# Autodesk Inventor assembly: X_CarriageR_V2_0_Short
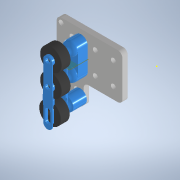
[picture p0: Inventor's stored thumbnail of the model, 180x180]
Saved by Autodesk Inventor 2021 (Build 250183000, 183)
## iProperties
Created: 2021-06-13
Part Number: X_CarriageR_V2_0_Short
Document SubType Name: Assembly
Designer: Jorian Brusind
Author: Jorian Brusind
## Documents named in this file (6)
- C:\Users\Jorian Bruslind\Documents\GitHub\PersonalProjects\HyperRail\Inventor Files\X_CarriageR_V2_0_Short.iam
- C:\Users\Jorian Bruslind\Documents\GitHub\PersonalProjects\HyperRail\Inventor Files\11mm_BearingWheel.ipt
- C:\Users\Jorian Bruslind\Documents\GitHub\PersonalProjects\HyperRail\Inventor Files\4mm_Roller_Spacer_simple.ipt
- C:\Users\Jorian Bruslind\Documents\GitHub\PersonalProjects\HyperRail\Inventor Files\Belt_Restraint.ipt
- C:\Users\Jorian Bruslind\Documents\GitHub\PersonalProjects\HyperRail\Inventor Files\Rollder_Spacer_Single.ipt
- C:\Users\Jorian Bruslind\Documents\GitHub\PersonalProjects\HyperRail\Inventor Files\X_Carriage_Plate_Short.ipt
## Components (8 placed, 5 different names)
1. 11mm_BearingWheel:2 — Flush:1, Mate:11, Mate:31
2. 11mm_BearingWheel:3 — Flush:1, Mate:12, Flush:4, Mate:32, Mate:33
3. 11mm_BearingWheel:5 — Flush:4, Mate:29, Mate:34
4. 4mm_Roller_Spacer_simple:1 — Mate:11, Mate:12, Mate:27, Mate:28, Mate:30, Mate:35, Mate:36
5. Belt_Restraint:1 — Mate:27, Mate:28, Mate:29, Mate:30
6. Belt_Restraint:2 — Mate:31, Mate:32, Mate:33
7. Rollder_Spacer_Single:1 — Mate:34, Mate:37
8. X_Carriage_Plate_Short:1 — Mate:35, Mate:36, Mate:37
## Relationships (15: Mate 13, Flush 2)
- Flush:1: 11mm_BearingWheel:2 ↔ 11mm_BearingWheel:3
- Mate:11: 11mm_BearingWheel:2 ↔ 4mm_Roller_Spacer_simple:1
- Mate:12: 11mm_BearingWheel:3 ↔ 4mm_Roller_Spacer_simple:1
- Flush:4: 11mm_BearingWheel:3 ↔ 11mm_BearingWheel:5
- Mate:27: 4mm_Roller_Spacer_simple:1 ↔ Belt_Restraint:1
- Mate:28: 4mm_Roller_Spacer_simple:1 ↔ Belt_Restraint:1
- Mate:29: 11mm_BearingWheel:5 ↔ Belt_Restraint:1
- Mate:30: 4mm_Roller_Spacer_simple:1 ↔ Belt_Restraint:1
- Mate:31: 11mm_BearingWheel:2 ↔ Belt_Restraint:2
- Mate:32: 11mm_BearingWheel:3 ↔ Belt_Restraint:2
- Mate:33: 11mm_BearingWheel:3 ↔ Belt_Restraint:2
- Mate:34: 11mm_BearingWheel:5 ↔ Rollder_Spacer_Single:1
- Mate:35: 4mm_Roller_Spacer_simple:1 ↔ X_Carriage_Plate_Short:1
- Mate:36: 4mm_Roller_Spacer_simple:1 ↔ X_Carriage_Plate_Short:1
- Mate:37: Rollder_Spacer_Single:1 ↔ X_Carriage_Plate_Short:1
